# Autodesk Inventor assembly: X Axis
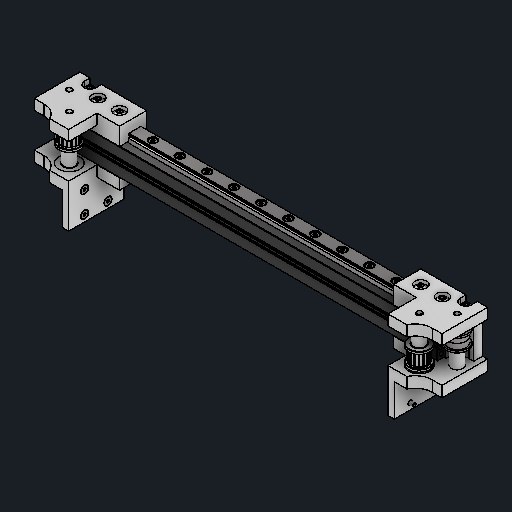
[picture p0: Inventor's stored thumbnail of the model, 512x512]
Saved by Autodesk Inventor 2026.2 (Build 302298000, 298)
## iProperties
Created: 2025-05-09
Part Number: X Axis
Document SubType Name: Assembly
Designer: AdminForWorker
Title: X Axis
Author: AdminForWorker
## Documents named in this file (6)
- C:\Users\JoshuaEah\Documents\GitHub\Voron-0\CAD\X Axis\X Axis.iam
- C:\Users\JoshuaEah\Documents\GitHub\Voron-0\CAD\Hardware\Linear Rail\MGN7 Rail 150mm.iam
- MGN7 150mm Rail.iam
- C:\Users\JoshuaEah\Documents\GitHub\Voron-0\CAD\Frame\Parts\1515 200mm - A.ipt
- C:\Users\JoshuaEah\Documents\GitHub\Voron-0\CAD\X Axis\XY Joints\XY Joint Left\XY Joint Left.iam
- C:\Users\JoshuaEah\Documents\GitHub\Voron-0\CAD\X Axis\XY Joints\XY Joint Right\XY Joint Right.iam
## Components (4 placed, 4 different names)
1. 1515 200mm - A (1):1 — Mate:1, Mate:2, Mate:3, Flush:1, Mate:4, Flush:2
2. MGN7 150mm Rail:1 [sub-assembly] — Mate:1, Mate:2, Mate:5, Mate:6
3. XY Joint Left:1 [sub-assembly] — Mate:3, Flush:1, Mate:6
4. XY Joint Right:1 [sub-assembly] — Mate:4, Flush:2, Mate:5
## Relationships (8: Mate 6, Flush 2)
- Mate:1 (0.1 mm): 1515 200mm - A (1):1 ↔ MGN7 150mm Rail:1
- Mate:2: 1515 200mm - A (1):1 ↔ MGN7 150mm Rail:1
- Mate:3: 1515 200mm - A (1):1 ↔ XY Joint Left:1
- Flush:1: 1515 200mm - A (1):1 ↔ XY Joint Left:1
- Mate:4: 1515 200mm - A (1):1 ↔ XY Joint Right:1
- Flush:2: 1515 200mm - A (1):1 ↔ XY Joint Right:1
- Mate:5 (1 mm): MGN7 150mm Rail:1 ↔ XY Joint Right:1
- Mate:6 (1 mm): MGN7 150mm Rail:1 ↔ XY Joint Left:1
